# Autodesk Inventor assembly: use this - gimme that tech award
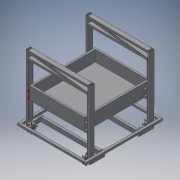
[picture p0: Inventor's stored thumbnail of the model, 180x180]
Saved by Autodesk Inventor 2018 (Build 220112000, 112)
## iProperties
Created: 2019-01-10
Part Number: use this - gimme that tech award
Document SubType Name: Assembly
Designer: maste
Author: maste
## Documents named in this file (8)
- C:\Users\maste\OneDrive\Documents\GitHub\2019CAD\Drivebase but Calvin is a mad man\use this - gimme that tech award.iam
- C:\Users\maste\OneDrive\Documents\GitHub\2019CAD\Drivebase but Calvin is a mad man\Slidey Mecanum L thing V2.iam
- C:\Users\maste\OneDrive\Documents\GitHub\2019CAD\Drivebase but Calvin is a mad man\Temporary Guide.ipt
- C:\Users\maste\OneDrive\Documents\GitHub\2019CAD\Drivebase but Calvin is a mad man\Temporary Platform.ipt
- C:\Users\maste\OneDrive\Documents\GitHub\2019CAD\Drivebase but Calvin is a mad man\1x1 30in.ipt
- C:\Users\maste\OneDrive\Documents\GitHub\2019CAD\Drivebase but Calvin is a mad man\1x1 35in.ipt
- C:\Users\maste\OneDrive\Documents\GitHub\2019CAD\Drivebase but Calvin is a mad man\1x1 L brackets 2in.ipt
- C:\Users\maste\OneDrive\Documents\GitHub\2019CAD\Drivebase but Calvin is a mad man\98404A101_18-8 STAINLESS STEEL QUICK-RELEASE PIN.ipt
## Components (19 placed, 7 different names)
1. Slidey Mecanum L thing V2:1 [sub-assembly] — Mate:17, Flush:16, Mate:18, Flush:17, Mate:29, Mate:30, Flush:20, Flush:22, Flush:24
2. Slidey Mecanum L thing V2:2 [sub-assembly] — Mate:19, Flush:18, Mate:20, Flush:19, Flush:21, Mate:42, Flush:23
3. Temporary Guide:1 — Mate:20, Flush:19, Mate:28
4. Temporary Guide:2 — Mate:18, Flush:17, Mate:24
5. Temporary Guide:3 — Mate:17, Flush:16, Mate:21, Mate:22, Mate:23
6. Temporary Guide:4 — Mate:19, Flush:18, Mate:25, Mate:26, Mate:27
7. Temporary Platform:1 — Mate:21, Mate:22, Mate:23, Mate:24, Mate:25, Mate:26, Mate:27, Mate:28
8. 1x1 30in:1 — Mate:31, Mate:32, Mate:33, Mate:34, Mate:35, Mate:36
9. 1x1 30in:2 — Mate:37, Mate:38, Mate:39
10. 1x1 35in:1 — Mate:29, Mate:30, Flush:20, Mate:31, Mate:32, Mate:33, Mate:45, Mate:46, Mate:47, Mate:48
11. 1x1 35in:2 — Mate:34, Mate:35, Mate:36, Mate:37, Mate:38, Mate:39, Mate:40, Mate:41, Mate:42, Mate:43, Mate:44
12. 1x1 L brackets 2in:1 — Flush:22, Mate:43, Mate:44, Mate:50, Flush:27, Rotation:2
13. 1x1 L brackets 2in:2 — Mate:40, Mate:41, Flush:21, Mate:49, Flush:28, Rotation:1
14. 1x1 L brackets 2in:3 — Mate:45, Mate:46, Flush:23, Mate:52, Flush:25, Rotation:4
15. 1x1 L brackets 2in:4 — Mate:47, Mate:48, Flush:24, Mate:51, Flush:26, Rotation:3
16. 98404A101_18-8 STAINLESS STEEL QUICK-RELEASE PIN:1 — Mate:52, Flush:25, Rotation:4
17. 98404A101_18-8 STAINLESS STEEL QUICK-RELEASE PIN:2 — Mate:51, Flush:26, Rotation:3
18. 98404A101_18-8 STAINLESS STEEL QUICK-RELEASE PIN:3 — Mate:50, Flush:27, Rotation:2
19. 98404A101_18-8 STAINLESS STEEL QUICK-RELEASE PIN:4 — Mate:49, Flush:28, Rotation:1
## Relationships (53: Mate 36, Flush 13, RelateRotation 4)
- Mate:17: Slidey Mecanum L thing V2:1 ↔ Temporary Guide:3
- Flush:16 (-16.9164 mm): Slidey Mecanum L thing V2:1 ↔ Temporary Guide:3
- Mate:18: Slidey Mecanum L thing V2:1 ↔ Temporary Guide:2
- Flush:17 (-16.9164 mm): Slidey Mecanum L thing V2:1 ↔ Temporary Guide:2
- Mate:19: Slidey Mecanum L thing V2:2 ↔ Temporary Guide:4
- Flush:18 (-16.9164 mm): Slidey Mecanum L thing V2:2 ↔ Temporary Guide:4
- Mate:20: Slidey Mecanum L thing V2:2 ↔ Temporary Guide:1
- Flush:19 (-16.9164 mm): Slidey Mecanum L thing V2:2 ↔ Temporary Guide:1
- Mate:21: Temporary Guide:3 ↔ Temporary Platform:1
- Mate:22: Temporary Guide:3 ↔ Temporary Platform:1
- Mate:23: Temporary Guide:3 ↔ Temporary Platform:1
- Mate:24: Temporary Guide:2 ↔ Temporary Platform:1
- Mate:25: Temporary Guide:4 ↔ Temporary Platform:1
- Mate:26: Temporary Guide:4 ↔ Temporary Platform:1
- Mate:27: Temporary Guide:4 ↔ Temporary Platform:1
- Mate:28: Temporary Guide:1 ↔ Temporary Platform:1
- Mate:29: Slidey Mecanum L thing V2:1 ↔ 1x1 35in:1
- Mate:30: Slidey Mecanum L thing V2:1 ↔ 1x1 35in:1
- Flush:20 (-76.2 mm): Slidey Mecanum L thing V2:1 ↔ 1x1 35in:1
- Mate:31: 1x1 30in:1 ↔ 1x1 35in:1
- Mate:32: 1x1 30in:1 ↔ 1x1 35in:1
- Mate:33: 1x1 30in:1 ↔ 1x1 35in:1
- Mate:34: 1x1 30in:1 ↔ 1x1 35in:2
- Mate:35: 1x1 30in:1 ↔ 1x1 35in:2
- Mate:36: 1x1 30in:1 ↔ 1x1 35in:2
- Mate:37: 1x1 30in:2 ↔ 1x1 35in:2
- Mate:38: 1x1 30in:2 ↔ 1x1 35in:2
- Mate:39: 1x1 30in:2 ↔ 1x1 35in:2
- Mate:40: 1x1 35in:2 ↔ 1x1 L brackets 2in:2
- Mate:41: 1x1 35in:2 ↔ 1x1 L brackets 2in:2
- Flush:21: Slidey Mecanum L thing V2:2 ↔ 1x1 L brackets 2in:2
- Mate:42: Slidey Mecanum L thing V2:2 ↔ 1x1 35in:2
- Flush:22: Slidey Mecanum L thing V2:1 ↔ 1x1 L brackets 2in:1
- Mate:43: 1x1 35in:2 ↔ 1x1 L brackets 2in:1
- Mate:44: 1x1 35in:2 ↔ 1x1 L brackets 2in:1
- Mate:45: 1x1 35in:1 ↔ 1x1 L brackets 2in:3
- Mate:46: 1x1 35in:1 ↔ 1x1 L brackets 2in:3
- Flush:23: Slidey Mecanum L thing V2:2 ↔ 1x1 L brackets 2in:3
- Mate:47: 1x1 35in:1 ↔ 1x1 L brackets 2in:4
- Mate:48: 1x1 35in:1 ↔ 1x1 L brackets 2in:4
- Flush:24: Slidey Mecanum L thing V2:1 ↔ 1x1 L brackets 2in:4
- Mate:49: 1x1 L brackets 2in:2 ↔ 98404A101_18-8 STAINLESS STEEL QUICK-RELEASE PIN:4
- Mate:50: 1x1 L brackets 2in:1 ↔ 98404A101_18-8 STAINLESS STEEL QUICK-RELEASE PIN:3
- Mate:51: 1x1 L brackets 2in:4 ↔ 98404A101_18-8 STAINLESS STEEL QUICK-RELEASE PIN:2
- Mate:52: 1x1 L brackets 2in:3 ↔ 98404A101_18-8 STAINLESS STEEL QUICK-RELEASE PIN:1
- Flush:25 (-10.16 mm): 1x1 L brackets 2in:3 ↔ 98404A101_18-8 STAINLESS STEEL QUICK-RELEASE PIN:1
- Flush:26 (-10.16 mm): 1x1 L brackets 2in:4 ↔ 98404A101_18-8 STAINLESS STEEL QUICK-RELEASE PIN:2
- Flush:27 (-10.16 mm): 1x1 L brackets 2in:1 ↔ 98404A101_18-8 STAINLESS STEEL QUICK-RELEASE PIN:3
- Flush:28 (-10.16 mm): 1x1 L brackets 2in:2 ↔ 98404A101_18-8 STAINLESS STEEL QUICK-RELEASE PIN:4
- Rotation:1 [RelateRotation] (1 ul): 1x1 L brackets 2in:2 ↔ 98404A101_18-8 STAINLESS STEEL QUICK-RELEASE PIN:4
- Rotation:2 [RelateRotation] (1 ul): 1x1 L brackets 2in:1 ↔ 98404A101_18-8 STAINLESS STEEL QUICK-RELEASE PIN:3
- Rotation:3 [RelateRotation] (1 ul): 1x1 L brackets 2in:4 ↔ 98404A101_18-8 STAINLESS STEEL QUICK-RELEASE PIN:2
- Rotation:4 [RelateRotation] (1 ul): 1x1 L brackets 2in:3 ↔ 98404A101_18-8 STAINLESS STEEL QUICK-RELEASE PIN:1
